# Autodesk Inventor assembly: Catapult
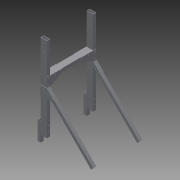
[picture p0: Inventor's stored thumbnail of the model, 180x180]
Saved by Autodesk Inventor 2013 (Build 170138000, 138)
## iProperties
Created: 2014-01-18
Part Number: Catapult
Document SubType Name: Assembly
Designer: 215152
Author: 215152
## Documents named in this file (7)
- D:\Robotics\FRC\2014\CAD\Robot\Catapult\Catapult.iam
- D:\Robotics\FRC\2014\CAD\Brian's Derp\Additions\SuperSuperStructure.ipt
- D:\Robotics\FRC\2014\CAD\Brian's Derp\Additions\CatapultGussetPlate.ipt
- D:\Robotics\FRC\2014\CAD\Brian's Derp\Additions\CatapultMotorSupport.ipt
- D:\Robotics\FRC\2014\CAD\Brian's Derp\Additions\SuperStructureSupport.ipt
- D:\Robotics\FRC\2014\CAD\Brian's Derp\Additions\SideSupport.ipt
- D:\Robotics\FRC\2014\CAD\Brian's Derp\Additions\SideGusset.ipt
## Components (13 placed, 6 different names)
1. SuperSuperStructure:1 — Mate:1, Flush:1, Flush:2, Mate:2, Mate:3, Flush:3, Mate:8, Flush:6, Mate:10, Mate:14, Flush:12, Mate:16, Mate:22, Flush:15, Mate:25, Flush:17, Mate:26
2. SuperSuperStructure:2 — Mate:1, Flush:1, Flush:2, Mate:4, Flush:4, Mate:6, Flush:5, Flush:7, Mate:12, Mate:13, Flush:11, Mate:15, Mate:21, Flush:14, Mate:23, Flush:16, Mate:24
3. CatapultGussetPlate:1 — Mate:2, Mate:3, Flush:3, Flush:8
4. CatapultGussetPlate:2 — Mate:6, Flush:5, Mate:11, Mate:12
5. CatapultGussetPlate:3 — Mate:8, Flush:6, Flush:9
6. CatapultGussetPlate:4 — Mate:4, Flush:4, Flush:10
7. CatapultMotorSupport:1 — Mate:10, Flush:7, Mate:11, Flush:8, Flush:9, Flush:10
8. SuperStructureSupport:1 — Mate:13, Flush:11, Mate:15
9. SuperStructureSupport:2 — Mate:14, Flush:12, Mate:16
10. SideSupport:1 — Mate:21, Flush:14, Flush:19
11. SideSupport:2 — Mate:22, Flush:15, Flush:20
12. SideGusset:1 — Mate:25, Flush:17, Mate:26, Flush:20
13. SideGusset:2 — Mate:23, Flush:16, Mate:24, Flush:19
## Relationships (37: Mate 19, Flush 18)
- Mate:1 (349.25 mm): SuperSuperStructure:1 ↔ SuperSuperStructure:2
- Flush:1: SuperSuperStructure:1 ↔ SuperSuperStructure:2
- Flush:2: SuperSuperStructure:1 ↔ SuperSuperStructure:2
- Mate:2: SuperSuperStructure:1 ↔ CatapultGussetPlate:1
- Mate:3: SuperSuperStructure:1 ↔ CatapultGussetPlate:1
- Flush:3: SuperSuperStructure:1 ↔ CatapultGussetPlate:1
- Mate:4: SuperSuperStructure:2 ↔ CatapultGussetPlate:4
- Flush:4: SuperSuperStructure:2 ↔ CatapultGussetPlate:4
- Mate:6: SuperSuperStructure:2 ↔ CatapultGussetPlate:2
- Flush:5: SuperSuperStructure:2 ↔ CatapultGussetPlate:2
- Mate:8: SuperSuperStructure:1 ↔ CatapultGussetPlate:3
- Flush:6: SuperSuperStructure:1 ↔ CatapultGussetPlate:3
- Mate:10: SuperSuperStructure:1 ↔ CatapultMotorSupport:1
- Flush:7: SuperSuperStructure:2 ↔ CatapultMotorSupport:1
- Mate:11: CatapultGussetPlate:2 ↔ CatapultMotorSupport:1
- Flush:8: CatapultGussetPlate:1 ↔ CatapultMotorSupport:1
- Flush:9: CatapultGussetPlate:3 ↔ CatapultMotorSupport:1
- Flush:10: CatapultGussetPlate:4 ↔ CatapultMotorSupport:1
- Mate:12: SuperSuperStructure:2 ↔ CatapultGussetPlate:2
- Mate:13: SuperSuperStructure:2 ↔ SuperStructureSupport:1
- Flush:11: SuperSuperStructure:2 ↔ SuperStructureSupport:1
- Mate:14: SuperSuperStructure:1 ↔ SuperStructureSupport:2
- Flush:12: SuperSuperStructure:1 ↔ SuperStructureSupport:2
- Mate:15: SuperSuperStructure:2 ↔ SuperStructureSupport:1
- Mate:16: SuperSuperStructure:1 ↔ SuperStructureSupport:2
- Mate:21: SuperSuperStructure:2 ↔ SideSupport:1
- Flush:14: SuperSuperStructure:2 ↔ SideSupport:1
- Mate:22: SuperSuperStructure:1 ↔ SideSupport:2
- Flush:15: SuperSuperStructure:1 ↔ SideSupport:2
- Mate:23: SuperSuperStructure:2 ↔ SideGusset:2
- Flush:16: SuperSuperStructure:2 ↔ SideGusset:2
- Mate:24: SuperSuperStructure:2 ↔ SideGusset:2
- Mate:25: SuperSuperStructure:1 ↔ SideGusset:1
- Flush:17: SuperSuperStructure:1 ↔ SideGusset:1
- Mate:26: SuperSuperStructure:1 ↔ SideGusset:1
- Flush:19: SideSupport:1 ↔ SideGusset:2
- Flush:20: SideSupport:2 ↔ SideGusset:1
